# Autodesk Inventor assembly: CapacitorBank.ipt
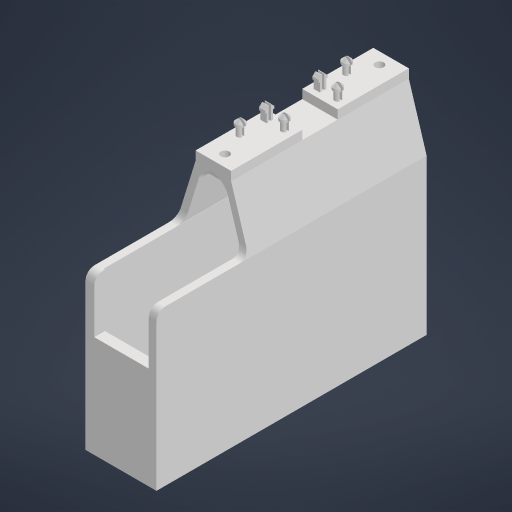
[picture p0: Inventor's stored thumbnail of the model, 512x512]
Saved by Autodesk Inventor 2024.1 (Build 281209000, 209)
## iProperties
Created: 2023-08-18
Part Number: CapacitorBank.ipt
Document SubType Name: Assembly
Designer: Eleanor
Author: Eleanor
## Documents named in this file (4)
- C:\Users\Eleanor\Documents\Inventor\4.5MM Electromanetic Rifle\CapacitorBank.ipt.iam
- C:\Users\Eleanor\Documents\Inventor\4.5MM Electromanetic Rifle\CapacitorBankDeck.ipt
- C:\Users\Eleanor\Documents\Inventor\4.5MM Electromanetic Rifle\MirrorBaseplate.ipt
- C:\Users\Eleanor\Documents\Inventor\4.5MM Electromanetic Rifle\MirrorBaseplate_MIR.ipt
## Components (3 placed, 3 different names)
1. CapacitorBankDeck:1 — Mate:3, Symmetry:1
2. MirrorBaseplate:2 — Mate:3, Symmetry:1
3. MirrorBaseplate_MIR:1
## Relationships (2: Mate 1, Symmetry 1)
- Mate:3: CapacitorBankDeck:1 ↔ MirrorBaseplate:2
- Symmetry:1: CapacitorBankDeck:1 ↔ MirrorBaseplate:2
